# Autodesk Inventor assembly: Thigh
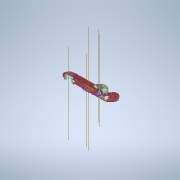
[picture p0: Inventor's stored thumbnail of the model, 180x180]
Saved by Autodesk Inventor 2022.2 (Build 262287000, 287)
## iProperties
Created: 2022-01-01
Part Number: Thigh
Document SubType Name: Assembly
Designer: Jochen
Author: Jochen
## Documents named in this file (10)
- D:\Projects\Chewbacca\CAD\Thigh\Thigh.iam
- D:\Projects\Chewbacca\CAD\Thigh\ThighBody.ipt
- D:\Projects\Chewbacca\CAD\Common\Encoder\encoder.iam
- D:\Projects\Chewbacca\CAD\Common\Motor\MotorModule.iam
- D:\Projects\Chewbacca\CAD\Common\Motor\Transmission Pulley.iam
- D:\Projects\Chewbacca\CAD\Thigh\Thigh\Design Accelerator\Synchronous Belts Transmission1.iam
- D:\Projects\Chewbacca\CAD\Common\Belt Tensioner\BeltTensioner 10mm.iam
- D:\Projects\Chewbacca\CAD\Common\Belt Tensioner\MotorBeltTensioner 10mm.iam
- D:\Projects\Chewbacca\CAD\Common\Motor\TransmissionPuileyCenter.iam
- D:\Projects\Chewbacca\CAD\Thigh\Thigh\Design Accelerator\Synchronous Belts Transmission2.iam
## Components (11 placed, 8 different names)
1. ThighBody V4:1 — Mate:1, Mate:2, Mate:3, Mate:4, Mate:5, Angle:1, Mate:6, Mate:7, Mate:14, Mate:15, Mate:16, Mate:23, Mate:28, Mate:29, Mate:31, Mate:32
2. Encoder:1 [sub-assembly] — Mate:3, Mate:5, Angle:1
3. MotorModule:1 [sub-assembly] — Mate:6, Mate:7, Mate:14
4. Transmission Pulley:1 [sub-assembly] — Mate:15, Mate:16
5. Synchronous Belts Transmission:1 [sub-assembly]
6. Belt tensioner 10mm:1 [sub-assembly]
7. Belt tensioner 10mm:2 [sub-assembly] — Mate:23
8. MotorBeltTensioner 10mm:1 [sub-assembly]
9. MotorBeltTensioner 10mm:2 [sub-assembly] — Mate:28, Mate:29
10. TransmissionPuleyCenter:1 [sub-assembly] — Mate:31, Mate:32
11. Synchronous Belts Transmission:2 [sub-assembly]
## Relationships (16: Mate 15, Angle 1)
- Mate:1: ThighBody V4:1
- Mate:2: ThighBody V4:1
- Mate:3: ThighBody V4:1 ↔ Encoder:1
- Mate:4: ThighBody V4:1
- Mate:5: ThighBody V4:1 ↔ Encoder:1
- Angle:1 (0 deg): ThighBody V4:1 ↔ Encoder:1
- Mate:6: ThighBody V4:1 ↔ MotorModule:1
- Mate:7: ThighBody V4:1 ↔ MotorModule:1
- Mate:14: ThighBody V4:1 ↔ MotorModule:1
- Mate:15: ThighBody V4:1 ↔ Transmission Pulley:1
- Mate:16: ThighBody V4:1 ↔ Transmission Pulley:1
- Mate:23: ThighBody V4:1 ↔ Belt tensioner 10mm:2
- Mate:28: ThighBody V4:1 ↔ MotorBeltTensioner 10mm:2
- Mate:29: ThighBody V4:1 ↔ MotorBeltTensioner 10mm:2
- Mate:31: ThighBody V4:1 ↔ TransmissionPuleyCenter:1
- Mate:32: ThighBody V4:1 ↔ TransmissionPuleyCenter:1
